# Autodesk Inventor assembly: Ankle_side_pitch
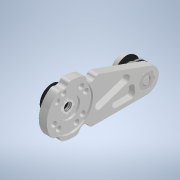
[picture p0: Inventor's stored thumbnail of the model, 180x180]
Saved by Autodesk Inventor 2020 (Build 240168000, 168)
## iProperties
Created: 2021-10-01
Part Number: Ankle_side_pitch
Document SubType Name: Assembly
Designer: Masato
Author: Masato
## Documents named in this file (8)
- C:\Users\Masato\Documents\Inventor\CIT Brains_Inventor\OpenPlatform_ver3_0\LowerBody\Ankle\Ankle_side_pitch.iam
- C:\Users\Masato\Documents\Inventor\CIT Brains_Inventor\OpenPlatform_ver3_0\LowerBody\Ankle\Ankle_side_pitch_frame.ipt
- C:\Users\Masato\Documents\Inventor\CIT Brains_Inventor\OpenPlatform_ver3_0\Ready_Made\80F-0603.ipt
- C:\Users\Masato\Documents\Inventor\CIT Brains_Inventor\OpenPlatform_ver3_0\Ready_Made\S4-07-3W.ipt
- C:\Users\Masato\Documents\Inventor\CIT Brains_Inventor\OpenPlatform_ver3_0\Ready_Made\SF419.ipt
- C:\Users\Masato\Documents\Inventor\CIT Brains_Inventor\OpenPlatform_ver3_0\Ready_Made\UUW-0412-10BH.ipt
- C:\Users\Masato\Documents\Inventor\CIT Brains_Inventor\OpenPlatform_ver3_0\Ready_Made\UUW-0612-05BH.ipt
- C:\Users\Masato\Documents\Inventor\CIT Brains_Inventor\OpenPlatform_ver3_0\Ready_Made\DBS4-5-5.ipt
## Components (10 placed, 7 different names)
1. Ankle_side_pitch_frame:1 — フラッシュ:2, メイト:1, 角度:1, 挿入:1, 挿入:2, 挿入:3, 挿入:4
2. 80F-0603:1 — 挿入:5
3. 80F-0603:2 — 挿入:6
4. S4-07-3W:1 — 角度:1, 挿入:1
5. SF419:1 — 挿入:2
6. UUW-0412-10BH:1 — 挿入:4, 挿入:5, 挿入:9
7. UUW-0412-10BH:2 — 挿入:3, 挿入:6
8. UUW-0612-05BH:1 — 挿入:7
9. UUW-0612-05BH:2
10. DBS4-5-5:1 — 挿入:9, 挿入:7
## Relationships (11: Insert 8, Flush 1, Mate 1, Angle 1)
- フラッシュ:2 [Flush]: Ankle_side_pitch_frame:1
- メイト:1 [Mate]: Ankle_side_pitch_frame:1
- 角度:1 [Angle] (0 deg): Ankle_side_pitch_frame:1 ↔ S4-07-3W:1
- 挿入:1 [Insert]: Ankle_side_pitch_frame:1 ↔ S4-07-3W:1
- 挿入:2 [Insert]: Ankle_side_pitch_frame:1 ↔ SF419:1
- 挿入:3 [Insert]: Ankle_side_pitch_frame:1 ↔ UUW-0412-10BH:2
- 挿入:4 [Insert]: Ankle_side_pitch_frame:1 ↔ UUW-0412-10BH:1
- 挿入:5 [Insert]: 80F-0603:1 ↔ UUW-0412-10BH:1
- 挿入:6 [Insert]: 80F-0603:2 ↔ UUW-0412-10BH:2
- 挿入:7 [Insert]: UUW-0612-05BH:1 ↔ DBS4-5-5:1
- 挿入:9 [Insert]: UUW-0412-10BH:1 ↔ DBS4-5-5:1
